# Autodesk Inventor assembly: 300-01
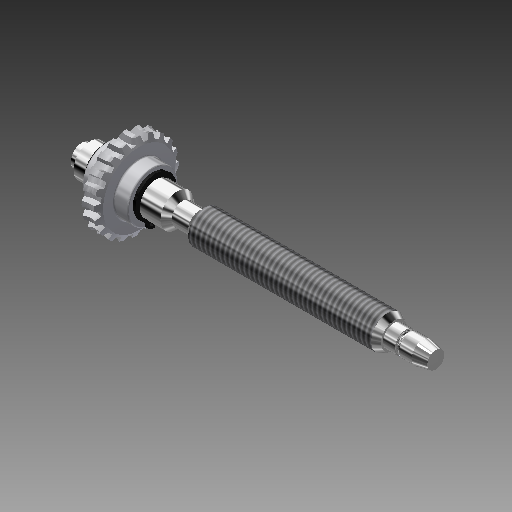
[picture p0: Inventor's stored thumbnail of the model, 512x512]
Saved by Autodesk Inventor 2019 (Build 230136000, 136)
## iProperties
Company: Autodesk Inc.
Created: 2007-12-26
Part Number: 300-01
Document SubType Name: Assembly
Designer: Autodesk Inc.
Mass: 108.136 g
Surface Area: 82.632 cm^2
Volume: 17.3544 cm^3
Density: 6.23103 g/cm^3
Description: BALL SCREW SHAFT ASSEMBLY
Component Category: Lower Component
Author: Inventor
## Documents named in this file (4)
- C:\TEMP\Car Seat\Workspace\Rear Ball Screw Shaft Assembly.iam
- C:\TEMP\Car Seat\Workspace\Worm Gear 20.ipt
- C:\TEMP\Car Seat\Workspace\Ball Screw Shaft A.ipt
- C:\TEMP\Car Seat\Workspace\JIS B 2804 12x1.ipt
## Components (4 placed, 3 different names)
1. Worm Gear:1 — Mate:1, Angle:1, Flush:1, Insert:1, Insert:3, Mate:2
2. Shaft:1 — Mate:1, Angle:1, Flush:1, Insert:2, Angle:2, Angle:3, Insert:3, Mate:2
3. JIS B 2804 12x1:1 — Insert:1, Angle:3
4. JIS B 2804 12x1:2 — Insert:2, Angle:2
## Relationships (9: Angle 3, Insert 3, Mate 2, Flush 1)
- Mate:1: Worm Gear:1 ↔ Shaft:1
- Angle:1 (180 deg): Worm Gear:1 ↔ Shaft:1
- Flush:1: Worm Gear:1 ↔ Shaft:1
- Insert:1: Worm Gear:1 ↔ JIS B 2804 12x1:1
- Insert:2: Shaft:1 ↔ JIS B 2804 12x1:2
- Angle:2 (270 deg): Shaft:1 ↔ JIS B 2804 12x1:2
- Angle:3 (90 deg): Shaft:1 ↔ JIS B 2804 12x1:1
- Insert:3: Worm Gear:1 ↔ Shaft:1
- Mate:2: Worm Gear:1 ↔ Shaft:1
